# Autodesk Inventor assembly: OdomHub
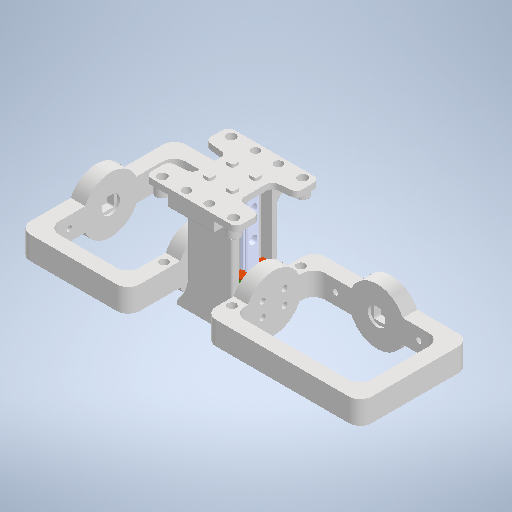
[picture p0: Inventor's stored thumbnail of the model, 512x512]
Saved by Autodesk Inventor 2025.1 (Build 291241020, 241B)
## iProperties
Created: 2025-02-12
Part Number: OdomHub
Document SubType Name: Assembly
Designer: AtuStem
Author: AtuStem
## Documents named in this file (6)
- C:\Users\AtuStem\Documents\GitHub\ATUM-V5RC-High-Stakes-CAD\Odometers_Collin\OdomHub.iam
- C:\Users\AtuStem\Documents\GitHub\ATUM-V5RC-High-Stakes-CAD\Odometers_Collin\Odom_Mega.ipt
- C:\Users\AtuStem\Documents\GitHub\ATUM-V5RC-High-Stakes-CAD\Odometers_Collin\Linear Rail Files\LinearRail-LWL7B-100mm\LinearRail-LWL7B-100mm\LinearRail-LWL7B-100mm.ipt
- C:\Users\AtuStem\Documents\GitHub\ATUM-V5RC-High-Stakes-CAD\Odometers_Collin\Linear Rail Files\Carriage-LWL7B\Carriage-LWL7B\Carriage-LWL7B.ipt
- C:\Users\AtuStem\Documents\GitHub\ATUM-V5RC-High-Stakes-CAD\Odometers_Collin\Linear_Odom.ipt
- C:\Users\AtuStem\Documents\GitHub\ATUM-V5RC-High-Stakes-CAD\Odometers_Collin\TheLongWay.ipt
## Components (7 placed, 5 different names)
1. Odom_Mega:1 — Mate:1, Mate:2, Mate:3, Mate:4, Mate:5, Mate:6, Mate:9, Mate:12
2. LinearRail-LWL7B-100mm:1 — Mate:1, Mate:4, Mate:5, Mate:10, Mate:11
3. LinearRail-LWL7B-100mm:2 — Mate:2, Mate:3, Mate:6, Mate:7, Mate:8
4. Carriage-LWL7B:3 — Mate:7, Mate:8, Mate:9, Mate:13, Mate:14, Mate:15
5. Carriage-LWL7B:4 — Mate:10, Mate:11, Mate:12, Mate:16, Mate:17, Mate:18
6. Linear_Odom:1 — Mate:13, Mate:14, Mate:15
7. TheLongWay:1 — Mate:16, Mate:17, Mate:18
## Relationships (18: Mate 18)
- Mate:1: Odom_Mega:1 ↔ LinearRail-LWL7B-100mm:1
- Mate:2: Odom_Mega:1 ↔ LinearRail-LWL7B-100mm:2
- Mate:3: Odom_Mega:1 ↔ LinearRail-LWL7B-100mm:2
- Mate:4: Odom_Mega:1 ↔ LinearRail-LWL7B-100mm:1
- Mate:5: Odom_Mega:1 ↔ LinearRail-LWL7B-100mm:1
- Mate:6: Odom_Mega:1 ↔ LinearRail-LWL7B-100mm:2
- Mate:7 (0.0762 mm): LinearRail-LWL7B-100mm:2 ↔ Carriage-LWL7B:3
- Mate:8 (0.1981 mm): LinearRail-LWL7B-100mm:2 ↔ Carriage-LWL7B:3
- Mate:9: Odom_Mega:1 ↔ Carriage-LWL7B:3
- Mate:10 (0.0762 mm): LinearRail-LWL7B-100mm:1 ↔ Carriage-LWL7B:4
- Mate:11 (0.1981 mm): LinearRail-LWL7B-100mm:1 ↔ Carriage-LWL7B:4
- Mate:12: Odom_Mega:1 ↔ Carriage-LWL7B:4
- Mate:13: Carriage-LWL7B:3 ↔ Linear_Odom:1
- Mate:14: Carriage-LWL7B:3 ↔ Linear_Odom:1
- Mate:15: Carriage-LWL7B:3 ↔ Linear_Odom:1
- Mate:16: Carriage-LWL7B:4 ↔ TheLongWay:1
- Mate:17: Carriage-LWL7B:4 ↔ TheLongWay:1
- Mate:18: Carriage-LWL7B:4 ↔ TheLongWay:1
